# Autodesk Inventor assembly: Chassis Assembly 26x28 Version
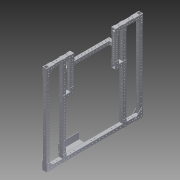
[picture p0: Inventor's stored thumbnail of the model, 180x180]
Saved by Autodesk Inventor 2013 (Build 170138000, 138)
## iProperties
Created: 2013-01-06
Part Number: Chassis Assembly 26x28 Version
Document SubType Name: Assembly
Designer: Moses
Mass: 3873.8 g
Surface Area: 9737.98 cm^2
Volume: 1429.45 cm^3
Density: 2.71 g/cm^3
Author: Moses
## Documents named in this file (13)
- C:\Users\Arpan\Documents\GitHub\frc2013CAD\Chassis\Chassis Assembly 26x28 Version\Chassis Assembly 26x28 Version.iam
- C:\Users\Arpan\Documents\GitHub\frc2013CAD\Chassis\Chassis V1.500 Part3-mirror.ipt
- C:\Users\Arpan\Documents\GitHub\frc2013CAD\Chassis\Chassis V1.500 Part2.ipt
- C:\Users\Arpan\Documents\GitHub\frc2013CAD\Chassis\Chassis V1.500 Part3.ipt
- C:\Users\Arpan\Documents\GitHub\frc2013CAD\Chassis\Chassis Connector Plate V1.500.ipt
- C:\Users\Arpan\Documents\GitHub\frc2013CAD\Chassis\Chassis Corner Plate V1.500.ipt
- C:\Users\Arpan\Documents\GitHub\frc2013CAD\Chassis\Chassis Assembly 26x28 Version\Chassis Part4 (26x28).ipt
- C:\Users\Arpan\Documents\GitHub\frc2013CAD\Chassis\Chassis Assembly 26x28 Version\Chassis Part1 (26x28).ipt
- C:\Users\Arpan\Documents\GitHub\frc2013CAD\Chassis\Chassis Assembly 26x28 Version\Chassis Battery Mount Part1.ipt
- C:\Users\Arpan\Documents\GitHub\frc2013CAD\Chassis\Chassis Assembly 26x28 Version\Chassis Part9 (26x28).ipt
- C:\Users\Arpan\Documents\GitHub\frc2013CAD\Chassis\Chassis Assembly 26x28 Version\Chassis Part10 (26x28).ipt
- C:\Users\Arpan\Documents\GitHub\frc2013CAD\Chassis\Chassis Assembly 26x28 Version\Chassis Part 11 (26x28).ipt
- C:\Users\Arpan\Documents\GitHub\frc2013CAD\Chassis\Chassis Assembly 26x28 Version\Chassis Part 12 (26x28).ipt
## Components (43 placed, 12 different names)
1. Chassis Part1 (26x28):1 — Mate:2, Flush:3, Flush:4, Flush:12, Mate:6, Flush:21, Flush:22, Mate:14, Flush:23, Flush:24, Mate:15, Flush:26, Mate:16, Flush:27, Flush:28, Flush:25
2. Chassis Part1 (26x28):2 — Mate:3, Flush:5, Flush:6, Flush:10, Mate:5, Flush:17, Mate:17, Flush:29, Flush:30, Mate:18, Flush:31, Flush:32, Mate:19, Flush:33, Flush:34, Mate:20, Flush:35, Flush:36
3. Chassis V1.500 Part2:1 — Mate:2, Flush:3, Flush:4, Mate:3, Flush:5, Flush:6, Mate:8, Mate:9, Flush:15, Flush:16, Mate:36, Mate:37, Mate:39, Mate:40, Mate:76, Mate:77, Mate:78, Mate:121, Mate:122, Mate:124, Mate:125
4. Chassis Part4 (26x28):1 — Flush:10, Mate:4, Flush:13, Mate:8, Flush:16, Mate:35, Mate:38, Mate:115, Mate:116, Mate:123, Mate:135, Flush:52, Mate:136
5. Chassis Part4 (26x28):2 — Flush:12, Flush:14, Mate:7, Mate:9, Flush:15, Mate:41, Mate:44, Mate:126, Mate:127, Mate:128, Mate:143, Flush:53
6. Chassis V1.500 Part3-mirror:1 — Mate:4, Mate:5, Flush:13, Mate:33, Mate:34, Mate:54, Flush:43, Flush:44, Mate:61, Mate:117, Mate:120
7. Chassis V1.500 Part3:1 — Mate:6, Flush:14, Mate:7, Mate:13, Mate:42, Mate:43, Mate:55, Flush:45, Flush:46, Mate:64, Mate:129, Mate:132
8. Chassis Corner Plate V1.500:1 — Flush:21, Mate:13, Flush:22
9. Chassis Corner Plate V1.500:2 — Mate:14, Flush:23, Flush:24
10. Chassis Corner Plate V1.500:3 — Mate:15, Flush:25, Flush:26
11. Chassis Corner Plate V1.500:4 — Mate:16, Flush:27, Flush:28
12. Chassis Corner Plate V1.500:5 — Mate:17, Flush:29, Flush:30
13. Chassis Corner Plate V1.500:6 — Mate:18, Flush:31, Flush:32
14. Chassis Corner Plate V1.500:7 — Mate:19, Flush:33, Flush:34
15. Chassis Corner Plate V1.500:8 — Mate:20, Flush:35, Flush:36
16. Chassis Connector Plate V1.500:5 — Mate:33, Mate:34, Mate:35
17. Chassis Connector Plate V1.500:6 — Mate:36, Mate:37, Mate:38
18. Chassis Connector Plate V1.500:7 — Mate:39, Mate:40, Mate:41
19. Chassis Connector Plate V1.500:8 — Mate:42, Mate:43, Mate:44
20. Chassis Connector Plate V1.500:9 — Mate:136, Mate:137
21. Chassis Connector Plate V1.500:10 — Mate:138, Mate:139
22. Chassis Connector Plate V1.500:11 — Mate:144, Mate:145
23. Chassis Connector Plate V1.500:12 — Mate:146, Mate:147
24. Chassis Part9 (26x28):1 — Mate:54, Flush:43, Flush:44, Mate:59, Mate:60, Mate:68, Flush:47, Mate:70, Flush:48, Mate:118, Mate:119, Mate:142, Mate:151, Flush:54
25. Chassis Part9 (26x28):2 — Mate:55, Flush:45, Flush:46, Mate:62, Mate:63, Mate:72, Mate:74, Flush:49, Flush:50, Mate:130, Mate:131, Mate:134, Flush:51, Mate:150, Mate:152, Flush:57, Mate:153
26. Chassis Connector Plate V1.500:14 — Mate:59, Mate:60, Mate:61
27. Chassis Connector Plate V1.500:16 — Mate:62, Mate:63, Mate:64
28. Chassis Connector Plate V1.500:17 — Mate:68, Flush:47, Mate:140, Mate:142
29. Chassis Connector Plate V1.500:18 — Mate:70, Flush:48, Mate:141
30. Chassis Connector Plate V1.500:19 — Mate:72, Flush:50, Mate:148, Mate:150
31. Chassis Connector Plate V1.500:20 — Mate:74, Flush:49, Mate:149
32. Chassis Battery Mount Part1:1 — Mate:76, Mate:77, Mate:78
33. Chassis Connector Plate V1.500:21 — Mate:115, Mate:116, Mate:117
34. Chassis Connector Plate V1.500:22 — Mate:118, Mate:119, Mate:120
35. Chassis Connector Plate V1.500:23 — Mate:121, Mate:122, Mate:123
36. Chassis Connector Plate V1.500:24 — Mate:124, Mate:125, Mate:126
37. Chassis Connector Plate V1.500:25 — Mate:127, Mate:128, Mate:129
38. Chassis Connector Plate V1.500:26 — Mate:130, Mate:131, Mate:132
39. Chassis Part10 (26x28):1 — Mate:134, Flush:51, Flush:55, Flush:56, Mate:153
40. Chassis Part 11 (26x28):1 — Mate:135, Flush:52, Mate:137, Mate:138, Mate:139, Mate:140, Mate:141
41. Chassis Part 11 (26x28):2 — Mate:143, Mate:144, Mate:145, Mate:146, Mate:147, Flush:53, Mate:148, Mate:149
42. Chassis Part 12 (26x28):1 — Mate:151, Flush:54, Flush:55
43. Chassis Part 12 (26x28):2 — Mate:152, Flush:56, Flush:57
## Relationships (123: Mate 81, Flush 42)
- Mate:2: Chassis Part1 (26x28):1 ↔ Chassis V1.500 Part2:1
- Flush:3: Chassis Part1 (26x28):1 ↔ Chassis V1.500 Part2:1
- Flush:4: Chassis Part1 (26x28):1 ↔ Chassis V1.500 Part2:1
- Mate:3: Chassis Part1 (26x28):2 ↔ Chassis V1.500 Part2:1
- Flush:5: Chassis Part1 (26x28):2 ↔ Chassis V1.500 Part2:1
- Flush:6: Chassis Part1 (26x28):2 ↔ Chassis V1.500 Part2:1
- Flush:10 (-120.65 mm): Chassis Part1 (26x28):2 ↔ Chassis Part4 (26x28):1
- Flush:12 (-120.65 mm): Chassis Part1 (26x28):1 ↔ Chassis Part4 (26x28):2
- Mate:4: Chassis Part4 (26x28):1 ↔ Chassis V1.500 Part3-mirror:1
- Mate:5: Chassis Part1 (26x28):2 ↔ Chassis V1.500 Part3-mirror:1
- Flush:13: Chassis Part4 (26x28):1 ↔ Chassis V1.500 Part3-mirror:1
- Mate:6: Chassis Part1 (26x28):1 ↔ Chassis V1.500 Part3:1
- Flush:14: Chassis Part4 (26x28):2 ↔ Chassis V1.500 Part3:1
- Mate:7: Chassis Part4 (26x28):2 ↔ Chassis V1.500 Part3:1
- Mate:8: Chassis V1.500 Part2:1 ↔ Chassis Part4 (26x28):1
- Mate:9: Chassis V1.500 Part2:1 ↔ Chassis Part4 (26x28):2
- Flush:15: Chassis V1.500 Part2:1 ↔ Chassis Part4 (26x28):2
- Flush:16: Chassis V1.500 Part2:1 ↔ Chassis Part4 (26x28):1
- Flush:17 (330.2 mm): Chassis Part1 (26x28):2
- Flush:21: Chassis Part1 (26x28):1 ↔ Chassis Corner Plate V1.500:1
- Mate:13: Chassis V1.500 Part3:1 ↔ Chassis Corner Plate V1.500:1
- Flush:22: Chassis Part1 (26x28):1 ↔ Chassis Corner Plate V1.500:1
- Mate:14: Chassis Part1 (26x28):1 ↔ Chassis Corner Plate V1.500:2
- Flush:23: Chassis Part1 (26x28):1 ↔ Chassis Corner Plate V1.500:2
- Flush:24: Chassis Part1 (26x28):1 ↔ Chassis Corner Plate V1.500:2
- Mate:15: Chassis Part1 (26x28):1 ↔ Chassis Corner Plate V1.500:3
- Flush:25: Chassis Part1 (26x28):1 ↔ Chassis Corner Plate V1.500:3
- Flush:26: Chassis Part1 (26x28):1 ↔ Chassis Corner Plate V1.500:3
- Mate:16: Chassis Part1 (26x28):1 ↔ Chassis Corner Plate V1.500:4
- Flush:27: Chassis Part1 (26x28):1 ↔ Chassis Corner Plate V1.500:4
- Flush:28: Chassis Part1 (26x28):1 ↔ Chassis Corner Plate V1.500:4
- Mate:17: Chassis Part1 (26x28):2 ↔ Chassis Corner Plate V1.500:5
- Flush:29: Chassis Part1 (26x28):2 ↔ Chassis Corner Plate V1.500:5
- Flush:30: Chassis Part1 (26x28):2 ↔ Chassis Corner Plate V1.500:5
- Mate:18: Chassis Part1 (26x28):2 ↔ Chassis Corner Plate V1.500:6
- Flush:31: Chassis Part1 (26x28):2 ↔ Chassis Corner Plate V1.500:6
- Flush:32: Chassis Part1 (26x28):2 ↔ Chassis Corner Plate V1.500:6
- Mate:19: Chassis Part1 (26x28):2 ↔ Chassis Corner Plate V1.500:7
- Flush:33: Chassis Part1 (26x28):2 ↔ Chassis Corner Plate V1.500:7
- Flush:34: Chassis Part1 (26x28):2 ↔ Chassis Corner Plate V1.500:7
- Mate:20: Chassis Part1 (26x28):2 ↔ Chassis Corner Plate V1.500:8
- Flush:35: Chassis Part1 (26x28):2 ↔ Chassis Corner Plate V1.500:8
- Flush:36: Chassis Part1 (26x28):2 ↔ Chassis Corner Plate V1.500:8
- Mate:33: Chassis V1.500 Part3-mirror:1 ↔ Chassis Connector Plate V1.500:5
- Mate:34: Chassis V1.500 Part3-mirror:1 ↔ Chassis Connector Plate V1.500:5
- Mate:35: Chassis Part4 (26x28):1 ↔ Chassis Connector Plate V1.500:5
- Mate:36: Chassis V1.500 Part2:1 ↔ Chassis Connector Plate V1.500:6
- Mate:37: Chassis V1.500 Part2:1 ↔ Chassis Connector Plate V1.500:6
- Mate:38: Chassis Part4 (26x28):1 ↔ Chassis Connector Plate V1.500:6
- Mate:39: Chassis V1.500 Part2:1 ↔ Chassis Connector Plate V1.500:7
- Mate:40: Chassis V1.500 Part2:1 ↔ Chassis Connector Plate V1.500:7
- Mate:41: Chassis Part4 (26x28):2 ↔ Chassis Connector Plate V1.500:7
- Mate:42: Chassis V1.500 Part3:1 ↔ Chassis Connector Plate V1.500:8
- Mate:43: Chassis V1.500 Part3:1 ↔ Chassis Connector Plate V1.500:8
- Mate:44: Chassis Part4 (26x28):2 ↔ Chassis Connector Plate V1.500:8
- Mate:54: Chassis V1.500 Part3-mirror:1 ↔ Chassis Part9 (26x28):1
- Flush:43: Chassis V1.500 Part3-mirror:1 ↔ Chassis Part9 (26x28):1
- Flush:44: Chassis V1.500 Part3-mirror:1 ↔ Chassis Part9 (26x28):1
- Mate:55: Chassis V1.500 Part3:1 ↔ Chassis Part9 (26x28):2
- Flush:45: Chassis V1.500 Part3:1 ↔ Chassis Part9 (26x28):2
- Flush:46: Chassis V1.500 Part3:1 ↔ Chassis Part9 (26x28):2
- Mate:59: Chassis Part9 (26x28):1 ↔ Chassis Connector Plate V1.500:14
- Mate:60: Chassis Part9 (26x28):1 ↔ Chassis Connector Plate V1.500:14
- Mate:61: Chassis V1.500 Part3-mirror:1 ↔ Chassis Connector Plate V1.500:14
- Mate:62: Chassis Part9 (26x28):2 ↔ Chassis Connector Plate V1.500:16
- Mate:63: Chassis Part9 (26x28):2 ↔ Chassis Connector Plate V1.500:16
- Mate:64: Chassis V1.500 Part3:1 ↔ Chassis Connector Plate V1.500:16
- Mate:68: Chassis Part9 (26x28):1 ↔ Chassis Connector Plate V1.500:17
- Flush:47: Chassis Part9 (26x28):1 ↔ Chassis Connector Plate V1.500:17
- Mate:70: Chassis Part9 (26x28):1 ↔ Chassis Connector Plate V1.500:18
- Flush:48: Chassis Part9 (26x28):1 ↔ Chassis Connector Plate V1.500:18
- Mate:72: Chassis Part9 (26x28):2 ↔ Chassis Connector Plate V1.500:19
- Mate:74: Chassis Part9 (26x28):2 ↔ Chassis Connector Plate V1.500:20
- Flush:49: Chassis Part9 (26x28):2 ↔ Chassis Connector Plate V1.500:20
- Flush:50: Chassis Part9 (26x28):2 ↔ Chassis Connector Plate V1.500:19
- Mate:76: Chassis V1.500 Part2:1 ↔ Chassis Battery Mount Part1:1
- Mate:77: Chassis V1.500 Part2:1 ↔ Chassis Battery Mount Part1:1
- Mate:78: Chassis V1.500 Part2:1 ↔ Chassis Battery Mount Part1:1
- Mate:115: Chassis Part4 (26x28):1 ↔ Chassis Connector Plate V1.500:21
- Mate:116: Chassis Part4 (26x28):1 ↔ Chassis Connector Plate V1.500:21
- Mate:117: Chassis V1.500 Part3-mirror:1 ↔ Chassis Connector Plate V1.500:21
- Mate:118: Chassis Part9 (26x28):1 ↔ Chassis Connector Plate V1.500:22
- Mate:119: Chassis Part9 (26x28):1 ↔ Chassis Connector Plate V1.500:22
- Mate:120: Chassis V1.500 Part3-mirror:1 ↔ Chassis Connector Plate V1.500:22
- Mate:121: Chassis V1.500 Part2:1 ↔ Chassis Connector Plate V1.500:23
- Mate:122: Chassis V1.500 Part2:1 ↔ Chassis Connector Plate V1.500:23
- Mate:123: Chassis Part4 (26x28):1 ↔ Chassis Connector Plate V1.500:23
- Mate:124: Chassis V1.500 Part2:1 ↔ Chassis Connector Plate V1.500:24
- Mate:125: Chassis V1.500 Part2:1 ↔ Chassis Connector Plate V1.500:24
- Mate:126: Chassis Part4 (26x28):2 ↔ Chassis Connector Plate V1.500:24
- Mate:127: Chassis Part4 (26x28):2 ↔ Chassis Connector Plate V1.500:25
- Mate:128: Chassis Part4 (26x28):2 ↔ Chassis Connector Plate V1.500:25
- Mate:129: Chassis V1.500 Part3:1 ↔ Chassis Connector Plate V1.500:25
- Mate:130: Chassis Part9 (26x28):2 ↔ Chassis Connector Plate V1.500:26
- Mate:131: Chassis Part9 (26x28):2 ↔ Chassis Connector Plate V1.500:26
- Mate:132: Chassis V1.500 Part3:1 ↔ Chassis Connector Plate V1.500:26
- Mate:134 (19.05 mm): Chassis Part9 (26x28):2 ↔ Chassis Part10 (26x28):1
- Flush:51: Chassis Part9 (26x28):2 ↔ Chassis Part10 (26x28):1
- Mate:135: Chassis Part4 (26x28):1 ↔ Chassis Part 11 (26x28):1
- Flush:52: Chassis Part4 (26x28):1 ↔ Chassis Part 11 (26x28):1
- Mate:136: Chassis Part4 (26x28):1 ↔ Chassis Connector Plate V1.500:9
- Mate:137: Chassis Connector Plate V1.500:9 ↔ Chassis Part 11 (26x28):1
- Mate:138: Chassis Connector Plate V1.500:10 ↔ Chassis Part 11 (26x28):1
- Mate:139: Chassis Connector Plate V1.500:10 ↔ Chassis Part 11 (26x28):1
- Mate:140: Chassis Connector Plate V1.500:17 ↔ Chassis Part 11 (26x28):1
- Mate:141: Chassis Connector Plate V1.500:18 ↔ Chassis Part 11 (26x28):1
- Mate:142: Chassis Part9 (26x28):1 ↔ Chassis Connector Plate V1.500:17
- Mate:143: Chassis Part4 (26x28):2 ↔ Chassis Part 11 (26x28):2
- Mate:144: Chassis Connector Plate V1.500:11 ↔ Chassis Part 11 (26x28):2
- Mate:145: Chassis Connector Plate V1.500:11 ↔ Chassis Part 11 (26x28):2
- Mate:146: Chassis Connector Plate V1.500:12 ↔ Chassis Part 11 (26x28):2
- Mate:147: Chassis Connector Plate V1.500:12 ↔ Chassis Part 11 (26x28):2
- Flush:53: Chassis Part4 (26x28):2 ↔ Chassis Part 11 (26x28):2
- Mate:148: Chassis Connector Plate V1.500:19 ↔ Chassis Part 11 (26x28):2
- Mate:149: Chassis Connector Plate V1.500:20 ↔ Chassis Part 11 (26x28):2
- Mate:150: Chassis Part9 (26x28):2 ↔ Chassis Connector Plate V1.500:19
- Mate:151: Chassis Part9 (26x28):1 ↔ Chassis Part 12 (26x28):1
- Flush:54: Chassis Part9 (26x28):1 ↔ Chassis Part 12 (26x28):1
- Flush:55: Chassis Part10 (26x28):1 ↔ Chassis Part 12 (26x28):1
- Mate:152: Chassis Part9 (26x28):2 ↔ Chassis Part 12 (26x28):2
- Flush:56: Chassis Part10 (26x28):1 ↔ Chassis Part 12 (26x28):2
- Flush:57: Chassis Part9 (26x28):2 ↔ Chassis Part 12 (26x28):2
- Mate:153: Chassis Part9 (26x28):2 ↔ Chassis Part10 (26x28):1
